# Autodesk Inventor assembly: Assembly
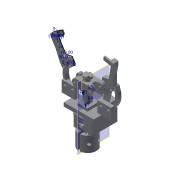
[picture p0: Inventor's stored thumbnail of the model, 180x180]
Saved by Autodesk Inventor 2018 (Build 220112000, 112)
## iProperties
Created: 2018-08-17
Part Number: Assembly
Document SubType Name: Assembly
Designer: Bardo91
Author: Bardo91
## Documents named in this file (9)
- E:\programming\hecatonquiros\cad_models\accesories\gripper_mini_screw\Assembly.iam
- E:\programming\hecatonquiros\cad_models\accesories\gripper_mini_screw\servoplace.ipt
- E:\programming\hecatonquiros\cad_models\accesories\servo_pwm_HD1160A.ipt
- E:\programming\hecatonquiros\cad_models\accesories\gripper_mini_screw\screw.ipt
- E:\programming\hecatonquiros\cad_models\accesories\gripper_mini_screw\screw_nut.ipt
- E:\programming\hecatonquiros\cad_models\accesories\gripper_mini_screw\bar_mid.ipt
- E:\programming\hecatonquiros\cad_models\accesories\gripper_mini_screw\bar_mid_2.ipt
- E:\programming\hecatonquiros\cad_models\accesories\gripper_mini_screw\gripper.ipt
- E:\programming\hecatonquiros\cad_models\accesories\gripper_mini_screw\tribar.ipt
## Components (11 placed, 8 different names)
1. servoplace:1 — Mate:1, Mate:2, Mate:3, Mate:8, Mate:9, Mate:12, Mate:13, Mate:14, Mate:15, Mate:16
2. servo_pwm_HD1160A:1 — Mate:1, Mate:2, Mate:3, Mate:4
3. screw:1 — Mate:4, Mate:5
4. screw_nut:1 — Mate:5, Mate:23, Mate:26
5. bar_mid:2 — Mate:12, Mate:19
6. bar_mid:4 — Mate:8, Mate:9, Mate:17, Mate:18
7. bar_mid_2:1 — Mate:13, Mate:14, Mate:22, Mate:25
8. bar_mid_2:2 — Mate:15, Mate:16
9. gripper:1 — Mate:17, Mate:18, Mate:21, Mate:24
10. gripper:2 — Mate:19
11. tribar:1 — Mate:21, Mate:22, Mate:23, Mate:24, Mate:25, Mate:26
## Relationships (21: Mate 21)
- Mate:1: servoplace:1 ↔ servo_pwm_HD1160A:1
- Mate:2: servoplace:1 ↔ servo_pwm_HD1160A:1
- Mate:3: servoplace:1 ↔ servo_pwm_HD1160A:1
- Mate:4: servo_pwm_HD1160A:1 ↔ screw:1
- Mate:5: screw:1 ↔ screw_nut:1
- Mate:8: servoplace:1 ↔ bar_mid:4
- Mate:9: servoplace:1 ↔ bar_mid:4
- Mate:12: servoplace:1 ↔ bar_mid:2
- Mate:13: servoplace:1 ↔ bar_mid_2:1
- Mate:14: servoplace:1 ↔ bar_mid_2:1
- Mate:15: servoplace:1 ↔ bar_mid_2:2
- Mate:16: servoplace:1 ↔ bar_mid_2:2
- Mate:17: bar_mid:4 ↔ gripper:1
- Mate:18: bar_mid:4 ↔ gripper:1
- Mate:19: bar_mid:2 ↔ gripper:2
- Mate:21: gripper:1 ↔ tribar:1
- Mate:22: bar_mid_2:1 ↔ tribar:1
- Mate:23: screw_nut:1 ↔ tribar:1
- Mate:24: gripper:1 ↔ tribar:1
- Mate:25: bar_mid_2:1 ↔ tribar:1
- Mate:26: screw_nut:1 ↔ tribar:1
